# Autodesk Inventor assembly: Propane Burner Assembly
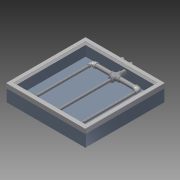
[picture p0: Inventor's stored thumbnail of the model, 180x180]
Saved by Autodesk Inventor 2013 SP2 (Build 170200200, 200)
## iProperties
Created: 2014-05-30
Part Number: Propane Burner Assembly
Document SubType Name: Assembly
Designer: jmw3
Author: jmw3
## Documents named in this file (10)
- F:\NIST\Propane Burner\Propane Burner Assembly.iam
- F:\NIST\Propane Burner\Propane Burner Base.ipt
- F:\NIST\Propane Burner\Propane Burner Lid.ipt
- F:\NIST\Propane Burner\Cross Pipe Fitting ASME B16.3 Class 150.ipt
- F:\NIST\Propane Burner\Welded Pipe Fitting ASTM A312 Schedule 40.ipt
- F:\NIST\Propane Burner\1 in pipe ASTM A 312 - Schedule 40S.ipt
- F:\NIST\Propane Burner\.5 in pipe.ipt
- F:\NIST\Propane Burner\.5 in pipe cap.ipt
- F:\NIST\Propane Burner\1 in to .5 in elbow reducer.ipt
- F:\NIST\Propane Burner\bushing.ipt
## Components (15 placed, 9 different names)
1. Propane Burner Base:1 — Mate:1, Mate:2, Mate:3, Mate:4, Flush:1, Rotation:1, Flush:3
2. Propane Burner Lid:1 — Mate:1, Mate:2, Mate:3
3. Cross Pipe Fitting ASME B16.3 Class 150:1 — Mate:44, Flush:2, Flush:4, Mate:45, Mate:46, Flush:5, Flush:9, Mate:55, Flush:16, Flush:17, Mate:57
4. Welded Pipe Fitting ASTM A312 Schedule 40:1 — Mate:4, Flush:1, Rotation:1, Mate:44, Flush:2
5. 1 in pipe ASTM A 312 - Schedule 40S:1 — Flush:8, Mate:51, Flush:9, Flush:10, Mate:52, Flush:11
6. .5 in pipe:1 — Mate:17, Rotation:8, Flush:12, Mate:53, Flush:13, Flush:14
7. .5 in pipe cap:1 — Mate:17, Rotation:8, Flush:14
8. .5 in pipe:2 — Mate:40, Mate:43, Rotation:18, Mate:56, Flush:17, Mate:57, Flush:18
9. .5 in pipe:3 — Mate:49, Mate:50, Flush:7, Mate:54, Flush:15
10. 1 in pipe ASTM A 312 - Schedule 40S:2 — Mate:45, Mate:46, Flush:5, Mate:47, Mate:48, Flush:6, Flush:8, Mate:51
11. .5 in pipe cap:4 — Mate:40, Mate:43, Rotation:18, Flush:18
12. .5 in pipe cap:5 — Mate:54, Flush:15
13. 1 in to .5 in elbow reducer:1 — Mate:47, Mate:48, Flush:6, Mate:49, Mate:50, Flush:7
14. 1 in to .5 in elbow reducer:2 — Flush:10, Mate:52, Flush:11, Flush:12, Mate:53, Flush:13
15. bushing:1 — Mate:55, Flush:16, Mate:56
## Relationships (42: Mate 21, Flush 18, RelateRotation 3)
- Mate:1: Propane Burner Base:1 ↔ Propane Burner Lid:1
- Mate:2: Propane Burner Base:1 ↔ Propane Burner Lid:1
- Mate:3: Propane Burner Base:1 ↔ Propane Burner Lid:1
- Mate:4: Propane Burner Base:1 ↔ Welded Pipe Fitting ASTM A312 Schedule 40:1
- Flush:1 (-25.4 mm): Propane Burner Base:1 ↔ Welded Pipe Fitting ASTM A312 Schedule 40:1
- Rotation:1 [RelateRotation] (1 ul): Propane Burner Base:1 ↔ Welded Pipe Fitting ASTM A312 Schedule 40:1
- Mate:17: .5 in pipe:1 ↔ .5 in pipe cap:1
- Rotation:8 [RelateRotation] (1.238 ul): .5 in pipe:1 ↔ .5 in pipe cap:1
- Mate:40: .5 in pipe:2 ↔ .5 in pipe cap:4
- Mate:43: .5 in pipe:2 ↔ .5 in pipe cap:4
- Rotation:18 [RelateRotation] (1.238 ul): .5 in pipe:2 ↔ .5 in pipe cap:4
- Mate:44: Cross Pipe Fitting ASME B16.3 Class 150:1 ↔ Welded Pipe Fitting ASTM A312 Schedule 40:1
- Flush:2: Cross Pipe Fitting ASME B16.3 Class 150:1 ↔ Welded Pipe Fitting ASTM A312 Schedule 40:1
- Flush:3: Propane Burner Base:1
- Flush:4: Cross Pipe Fitting ASME B16.3 Class 150:1
- Mate:45: Cross Pipe Fitting ASME B16.3 Class 150:1 ↔ 1 in pipe ASTM A 312 - Schedule 40S:2
- Mate:46: Cross Pipe Fitting ASME B16.3 Class 150:1 ↔ 1 in pipe ASTM A 312 - Schedule 40S:2
- Flush:5: Cross Pipe Fitting ASME B16.3 Class 150:1 ↔ 1 in pipe ASTM A 312 - Schedule 40S:2
- Mate:47: 1 in pipe ASTM A 312 - Schedule 40S:2 ↔ 1 in to .5 in elbow reducer:1
- Mate:48: 1 in pipe ASTM A 312 - Schedule 40S:2 ↔ 1 in to .5 in elbow reducer:1
- Flush:6: 1 in pipe ASTM A 312 - Schedule 40S:2 ↔ 1 in to .5 in elbow reducer:1
- Mate:49: .5 in pipe:3 ↔ 1 in to .5 in elbow reducer:1
- Mate:50: .5 in pipe:3 ↔ 1 in to .5 in elbow reducer:1
- Flush:7: .5 in pipe:3 ↔ 1 in to .5 in elbow reducer:1
- Flush:8: 1 in pipe ASTM A 312 - Schedule 40S:1 ↔ 1 in pipe ASTM A 312 - Schedule 40S:2
- Mate:51: 1 in pipe ASTM A 312 - Schedule 40S:1 ↔ 1 in pipe ASTM A 312 - Schedule 40S:2
- Flush:9: Cross Pipe Fitting ASME B16.3 Class 150:1 ↔ 1 in pipe ASTM A 312 - Schedule 40S:1
- Flush:10: 1 in pipe ASTM A 312 - Schedule 40S:1 ↔ 1 in to .5 in elbow reducer:2
- Mate:52: 1 in pipe ASTM A 312 - Schedule 40S:1 ↔ 1 in to .5 in elbow reducer:2
- Flush:11: 1 in pipe ASTM A 312 - Schedule 40S:1 ↔ 1 in to .5 in elbow reducer:2
- Flush:12: .5 in pipe:1 ↔ 1 in to .5 in elbow reducer:2
- Mate:53: .5 in pipe:1 ↔ 1 in to .5 in elbow reducer:2
- Flush:13: .5 in pipe:1 ↔ 1 in to .5 in elbow reducer:2
- Flush:14: .5 in pipe:1 ↔ .5 in pipe cap:1
- Mate:54: .5 in pipe:3 ↔ .5 in pipe cap:5
- Flush:15: .5 in pipe:3 ↔ .5 in pipe cap:5
- Mate:55: Cross Pipe Fitting ASME B16.3 Class 150:1 ↔ bushing:1
- Flush:16: Cross Pipe Fitting ASME B16.3 Class 150:1 ↔ bushing:1
- Mate:56: .5 in pipe:2 ↔ bushing:1
- Flush:17: Cross Pipe Fitting ASME B16.3 Class 150:1 ↔ .5 in pipe:2
- Mate:57: Cross Pipe Fitting ASME B16.3 Class 150:1 ↔ .5 in pipe:2
- Flush:18: .5 in pipe:2 ↔ .5 in pipe cap:4
